# Autodesk Inventor assembly: SensorSystem
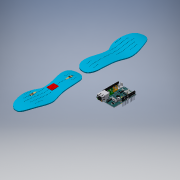
[picture p0: Inventor's stored thumbnail of the model, 180x180]
Saved by Autodesk Inventor 2016 (Build 200138000, 138)
## iProperties
Created: 2018-02-21
Part Number: SensorSystem
Document SubType Name: Assembly
Designer: Administrator
Author: Administrator
## Documents named in this file (5)
- F:\Dropbox\GaitDiagnosisML\InventorModel\Imported Components\SensorSystem.iam
- F:\Dropbox\GaitDiagnosisML\InventorModel\Imported Components\Arduino_Ethernet_Shield_V2.iam
- F:\Dropbox\GaitDiagnosisML\InventorModel\Imported Components\showinsole.ipt
- F:\Dropbox\GaitDiagnosisML\InventorModel\Imported Components\ForceSensor.iam
- F:\Dropbox\GaitDiagnosisML\InventorModel\Imported Components\IMU6dof.ipt
## Components (5 placed, 4 different names)
1. Arduino_Ethernet_Shield_V2:1 [sub-assembly]
2. showinsole:1 — Mate:2, Mate:3, Rigid:2, Rigid:3, Rigid:4
3. ForceSensor:1 [sub-assembly] — Rigid:2
4. ForceSensor:2 [sub-assembly] — Rigid:3
5. IMU6dof:1 — Rigid:4
## Relationships (5: WeldJoint 3, Mate 2)
- Mate:2 (76.2 mm): showinsole:1
- Mate:3 (-25.4 mm): showinsole:1
- Rigid:2 [WeldJoint] (-0.508 mm): showinsole:1 ↔ ForceSensor:1
- Rigid:3 [WeldJoint] (-0.762 mm): showinsole:1 ↔ ForceSensor:2
- Rigid:4 [WeldJoint] (-1.27 mm): showinsole:1 ↔ IMU6dof:1
